# Autodesk Inventor assembly: ASY MSC 080 gills
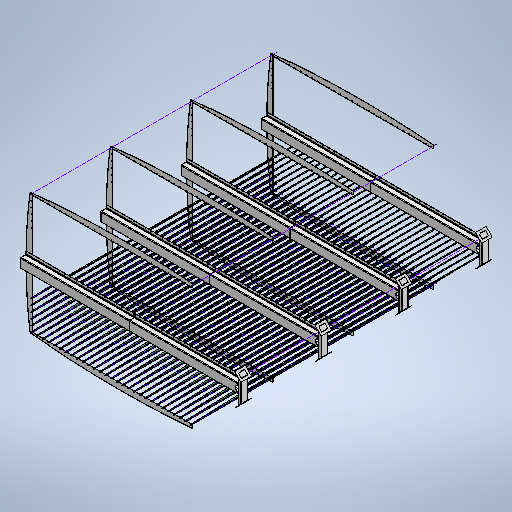
[picture p0: Inventor's stored thumbnail of the model, 512x512]
Saved by Autodesk Inventor 2025 (Build 290162010, 162A)
## iProperties
Created: 2024-08-31
Part Number: ASY MSC 080 gills
Document SubType Name: Assembly
Designer: pokla
Stock Number: ASY МОО 080 Жабры
Author: pokla
## Documents named in this file (20)
- C:\Users\admin\YandexDisk-badmisterfox\домашниий пк\Inventor\Manturovo\Manturovo_Se-clar\ASY MSC 080 gills.iam
- C:\Users\admin\YandexDisk-badmisterfox\домашниий пк\Inventor\Manturovo\Manturovo_Se-clar\MSC 802 sheet gills.ipt
- C:\Users\admin\YandexDisk-badmisterfox\домашниий пк\Inventor\Manturovo\Manturovo_Se-clar\MSC 081 pillar gills.ipt
- C:\Users\admin\YandexDisk-badmisterfox\домашниий пк\Inventor\Manturovo\Manturovo_Se-clar\MSC 804 sheet gills.ipt
- C:\Users\admin\YandexDisk-badmisterfox\домашниий пк\Inventor\Manturovo\Manturovo_Se-clar\MSC 803 sheet gills.ipt
- C:\Users\admin\YandexDisk-badmisterfox\домашниий пк\Inventor\Manturovo\Manturovo_Se-clar\MSC 806 sheet gills.ipt
- C:\Users\admin\YandexDisk-badmisterfox\домашниий пк\Inventor\Manturovo\Manturovo_Se-clar\MSC 805 sheet gills.ipt
- C:\Users\admin\YandexDisk-badmisterfox\домашниий пк\Inventor\Manturovo\Manturovo_Se-clar\MSC 808 sheet gills.ipt
- C:\Users\admin\YandexDisk-badmisterfox\домашниий пк\Inventor\Manturovo\Manturovo_Se-clar\MSC 807 sheet gills.ipt
- C:\Users\admin\YandexDisk-badmisterfox\домашниий пк\Inventor\Manturovo\Manturovo_Se-clar\MSC 810 sheet gills.ipt
- C:\Users\admin\YandexDisk-badmisterfox\домашниий пк\Inventor\Manturovo\Manturovo_Se-clar\MSC 809 sheet gills.ipt
- C:\Users\admin\YandexDisk-badmisterfox\домашниий пк\Inventor\Manturovo\Manturovo_Se-clar\MSC 812 sheet gills.ipt
- C:\Users\admin\YandexDisk-badmisterfox\домашниий пк\Inventor\Manturovo\Manturovo_Se-clar\MSC 811 sheet gills.ipt
- C:\Users\admin\YandexDisk-badmisterfox\домашниий пк\Inventor\Manturovo\Manturovo_Se-clar\MSC 084 wall support gills.ipt
- C:\Users\admin\YandexDisk-badmisterfox\домашниий пк\Inventor\Manturovo\Manturovo_Se-clar\MSC 085 bottom support gills.ipt
- C:\Users\admin\YandexDisk-badmisterfox\домашниий пк\Inventor\Manturovo\Manturovo_Se-clar\MSC 082 pillar gills.ipt
- C:\Users\admin\YandexDisk-badmisterfox\домашниий пк\Inventor\Manturovo\Manturovo_Se-clar\MSC 086 string for sheets gills.ipt
- C:\Users\admin\YandexDisk-badmisterfox\домашниий пк\Inventor\Manturovo\Manturovo_Se-clar\MSC 083 top support gills.ipt
- C:\Users\admin\YandexDisk-badmisterfox\домашниий пк\Inventor\Manturovo\Manturovo_Se-clar\MSC 087 bottom plate gills.ipt
- C:\Users\admin\YandexDisk-badmisterfox\домашниий пк\Inventor\Manturovo\Manturovo_Se-clar\MSC 801 sheet gills.ipt
## Components (175 placed, 19 different names)
1. MSC 804 sheet gills:1 — Rigid:39
2. MSC 803 sheet gills:1 — Angle:2, Tangent:8, Tangent:9, Flush:15, Flush:19, Rigid:39
3. MSC 806 sheet gills:1 — Rigid:36
4. MSC 805 sheet gills:1 — Rigid:36, Angle:3, Tangent:10, Tangent:11, Flush:15, Flush:16
5. MSC 808 sheet gills:1 — Rigid:37
6. MSC 807 sheet gills:1 — Rigid:37, Angle:4, Tangent:12, Tangent:13, Flush:16, Flush:17
7. MSC 810 sheet gills:1 — Rigid:38
8. MSC 809 sheet gills:1 — Rigid:38, Angle:5, Tangent:17, Tangent:18, Flush:17, Flush:18
9. MSC 812 sheet gills:1 — Rigid:32
10. MSC 811 sheet gills:1 — Rigid:32, Angle:6, Tangent:19, Tangent:20, Flush:18
11. MSC 084 wall support gills:1 — Rigid:12, Rigid:25, Rigid:30, Tangent:14, Tangent:15
12. MSC 084 wall support gills:2 — Rigid:25, Rigid:26, Mate:17
13. MSC 084 wall support gills:3 — Rigid:26, Rigid:27
14. MSC 084 wall support gills:4 — Rigid:27
15. MSC 086 string for sheets gills:2 — Rigid:15
16. MSC 086 string for sheets gills:57 — Rotational:2
17. MSC 085 bottom support gills:1 — Rigid:6, Rigid:7, Flush:12, Mate:12, Flush:14, Mate:15, Mate:16, Flush:9
18. MSC 081 pillar gills:1 — Flush:12, Mate:12, Flush:14, Rotational:1, Rotational:2, Tangent:16
19. MSC 082 pillar gills:1 — Rigid:28, Rigid:29
20. MSC 085 bottom support gills:2
21. MSC 081 pillar gills:2
22. MSC 082 pillar gills:2
23. MSC 085 bottom support gills:3
24. MSC 081 pillar gills:3
25. MSC 082 pillar gills:3
26. MSC 085 bottom support gills:4
27. MSC 081 pillar gills:4
28. MSC 082 pillar gills:4
29. MSC 801 sheet gills:1 — Mate:17, Rigid:33, Angle:2, Angle:3, Angle:4, Angle:5, Angle:6, Tangent:14, Tangent:15, Tangent:16, Flush:19
30. MSC 802 sheet gills:1 — Rigid:33
31. MSC 801 sheet gills:2
32. MSC 802 sheet gills:2
33. MSC 801 sheet gills:3
34. MSC 802 sheet gills:3
35. MSC 801 sheet gills:4
36. MSC 802 sheet gills:4
37. MSC 801 sheet gills:5
38. MSC 802 sheet gills:5
39. MSC 801 sheet gills:6
40. MSC 802 sheet gills:6
41. MSC 801 sheet gills:7
42. MSC 802 sheet gills:7
43. MSC 801 sheet gills:8
44. MSC 802 sheet gills:8
45. MSC 801 sheet gills:9
46. MSC 802 sheet gills:9
47. MSC 801 sheet gills:10
48. MSC 802 sheet gills:10
49. MSC 801 sheet gills:11
50. MSC 802 sheet gills:11
51. MSC 801 sheet gills:12
52. MSC 802 sheet gills:12
53. MSC 801 sheet gills:13
54. MSC 802 sheet gills:13
55. MSC 801 sheet gills:14
56. MSC 802 sheet gills:14
57. MSC 801 sheet gills:15
58. MSC 802 sheet gills:15
59. MSC 801 sheet gills:16
60. MSC 802 sheet gills:16
61. MSC 801 sheet gills:17
62. MSC 802 sheet gills:17
63. MSC 801 sheet gills:18
64. MSC 802 sheet gills:18
65. MSC 801 sheet gills:19
66. MSC 802 sheet gills:19
67. MSC 801 sheet gills:20
68. MSC 802 sheet gills:20
69. MSC 801 sheet gills:21
70. MSC 802 sheet gills:21
71. MSC 801 sheet gills:22
72. MSC 802 sheet gills:22
73. MSC 801 sheet gills:23
74. MSC 802 sheet gills:23
75. MSC 801 sheet gills:24
76. MSC 802 sheet gills:24
77. MSC 801 sheet gills:25
78. MSC 802 sheet gills:25
79. MSC 801 sheet gills:26
80. MSC 802 sheet gills:26
81. MSC 801 sheet gills:27
82. MSC 802 sheet gills:27
83. MSC 801 sheet gills:28
84. MSC 802 sheet gills:28
85. MSC 801 sheet gills:29
86. MSC 802 sheet gills:29
87. MSC 084 wall support gills:5 — Rigid:15, Rigid:31
88. MSC 083 top support gills:1 — Rigid:24, Rigid:29, Rigid:31
89. MSC 083 top support gills:2 — Rigid:28, Rigid:30, Tangent:8, Tangent:9, Tangent:10, Tangent:11, Tangent:12, Tangent:13, Tangent:17, Tangent:18, Tangent:19, Tangent:20, Rigid:40
90. MSC 087 bottom plate gills:1 — Rigid:6
91. MSC 087 bottom plate gills:2 — Rigid:7
92. MSC 084 wall support gills:6
93. MSC 083 top support gills:3
94. MSC 083 top support gills:4
95. MSC 087 bottom plate gills:3
96. MSC 087 bottom plate gills:4
97. MSC 084 wall support gills:7
98. MSC 083 top support gills:5
99. MSC 083 top support gills:6
100. MSC 087 bottom plate gills:5
101. MSC 087 bottom plate gills:6
102. MSC 084 wall support gills:8
103. MSC 083 top support gills:7
104. MSC 083 top support gills:8
105. MSC 087 bottom plate gills:7
106. MSC 087 bottom plate gills:8
107. MSC 086 string for sheets gills:1 — Rigid:12
108. MSC 086 string for sheets gills:3
109. MSC 086 string for sheets gills:5
110. MSC 086 string for sheets gills:7
111. MSC 086 string for sheets gills:9
112. MSC 086 string for sheets gills:11
113. MSC 086 string for sheets gills:13
114. MSC 086 string for sheets gills:15
115. MSC 086 string for sheets gills:17
116. MSC 086 string for sheets gills:19
117. MSC 086 string for sheets gills:21
118. MSC 086 string for sheets gills:23
119. MSC 086 string for sheets gills:25
120. MSC 086 string for sheets gills:27
121. MSC 086 string for sheets gills:29
122. MSC 086 string for sheets gills:31
123. MSC 086 string for sheets gills:33
124. MSC 086 string for sheets gills:35
125. MSC 086 string for sheets gills:37
126. MSC 086 string for sheets gills:39
127. MSC 086 string for sheets gills:41
128. MSC 086 string for sheets gills:43
129. MSC 086 string for sheets gills:45
130. MSC 086 string for sheets gills:47
131. MSC 086 string for sheets gills:49
132. MSC 086 string for sheets gills:51
133. MSC 086 string for sheets gills:53
134. MSC 086 string for sheets gills:55
135. MSC 086 string for sheets gills:58 — Rotational:1
136. MSC 086 string for sheets gills:60
137. MSC 086 string for sheets gills:62
138. MSC 086 string for sheets gills:64
139. MSC 086 string for sheets gills:66
140. MSC 086 string for sheets gills:68
141. MSC 086 string for sheets gills:70
142. MSC 086 string for sheets gills:72
143. MSC 086 string for sheets gills:74
144. MSC 086 string for sheets gills:76
145. MSC 086 string for sheets gills:78
146. MSC 086 string for sheets gills:80
147. MSC 086 string for sheets gills:82
148. MSC 086 string for sheets gills:84
149. MSC 086 string for sheets gills:86
150. MSC 086 string for sheets gills:88
151. MSC 086 string for sheets gills:90
152. MSC 086 string for sheets gills:92
153. MSC 086 string for sheets gills:94
154. MSC 086 string for sheets gills:96
155. MSC 086 string for sheets gills:98
156. MSC 086 string for sheets gills:100
157. MSC 086 string for sheets gills:102
158. MSC 086 string for sheets gills:104
159. MSC 086 string for sheets gills:106
160. MSC 086 string for sheets gills:108
161. MSC 086 string for sheets gills:110
162. MSC 086 string for sheets gills:112
163. MSC 086 string for sheets gills:114
164. MSC 086 string for sheets gills:116
165. MSC 086 string for sheets gills:118
166. MSC 086 string for sheets gills:120
167. MSC 086 string for sheets gills:122
168. MSC 086 string for sheets gills:124
169. MSC 086 string for sheets gills:125 — Rigid:40
170. MSC 086 string for sheets gills:126
171. MSC 086 string for sheets gills:127
172. MSC 086 string for sheets gills:128
173. MSC 086 string for sheets gills:129
174. MSC 086 string for sheets gills:130
175. MSC 086 string for sheets gills:131 — Rigid:24
## Component patterns: (4 elements, first: MSC 085 bottom support gills:1 + MSC 081 pillar gills:1 + MSC 082 pillar gills:1), (29 elements, first: MSC 801 sheet gills:1 + MSC 802 sheet gills:1), (4 elements, first: MSC 084 wall support gills:5 + MSC 083 top support gills:1 + MSC 083 top support gills:2 + MSC 087 bottom plate gills:1 + MSC 087 bottom plate gills:2), (28 elements, first: MSC 086 string for sheets gills:1), (34 elements, first: MSC 086 string for sheets gills:58), (6 elements, first: MSC 086 string for sheets gills:125), (1 elements, first: MSC 086 string for sheets gills:131)
## Relationships (52: WeldJoint 20, Tangent 13, Flush 8, Angle 5, Mate 4, RevoluteJoint 2)
- [WeldJoint]: MSC 081 pillar gills:1 ↔ MSC 082 pillar gills:1
- Rigid:6 [WeldJoint]: MSC 085 bottom support gills:1 ↔ MSC 087 bottom plate gills:1
- Rigid:7 [WeldJoint]: MSC 085 bottom support gills:1 ↔ MSC 087 bottom plate gills:2
- Flush:12: MSC 085 bottom support gills:1 ↔ MSC 081 pillar gills:1
- Mate:12: MSC 085 bottom support gills:1 ↔ MSC 081 pillar gills:1
- Flush:14 (5 mm): MSC 085 bottom support gills:1 ↔ MSC 081 pillar gills:1
- Rigid:12 [WeldJoint] (-5 mm): MSC 084 wall support gills:1 ↔ MSC 086 string for sheets gills:1
- Rigid:15 [WeldJoint] (-5 mm): MSC 086 string for sheets gills:2 ↔ MSC 084 wall support gills:5
- Mate:15: MSC 085 bottom support gills:1
- Mate:16: MSC 085 bottom support gills:1
- Flush:9: MSC 085 bottom support gills:1
- Rigid:24 [WeldJoint] (-5 mm): MSC 083 top support gills:1 ↔ MSC 086 string for sheets gills:131
- Rigid:25 [WeldJoint] (985 mm): MSC 084 wall support gills:1 ↔ MSC 084 wall support gills:2
- Rigid:26 [WeldJoint] (985 mm): MSC 084 wall support gills:2 ↔ MSC 084 wall support gills:3
- Rigid:27 [WeldJoint] (985 mm): MSC 084 wall support gills:3 ↔ MSC 084 wall support gills:4
- Mate:17: MSC 084 wall support gills:2 ↔ MSC 801 sheet gills:1
- Rigid:28 [WeldJoint]: MSC 082 pillar gills:1 ↔ MSC 083 top support gills:2
- Rigid:29 [WeldJoint]: MSC 082 pillar gills:1 ↔ MSC 083 top support gills:1
- Rigid:30 [WeldJoint]: MSC 084 wall support gills:1 ↔ MSC 083 top support gills:2
- Rigid:31 [WeldJoint]: MSC 084 wall support gills:5 ↔ MSC 083 top support gills:1
- Rotational:1 [RevoluteJoint] (5 mm): MSC 081 pillar gills:1 ↔ MSC 086 string for sheets gills:58
- Rotational:2 [RevoluteJoint] (-5 mm): MSC 086 string for sheets gills:57 ↔ MSC 081 pillar gills:1
- Rigid:32 [WeldJoint] (-10 mm): MSC 812 sheet gills:1 ↔ MSC 811 sheet gills:1
- Rigid:33 [WeldJoint] (-10 mm): MSC 801 sheet gills:1 ↔ MSC 802 sheet gills:1
- Rigid:36 [WeldJoint] (-10 mm): MSC 806 sheet gills:1 ↔ MSC 805 sheet gills:1
- Rigid:37 [WeldJoint] (-10 mm): MSC 808 sheet gills:1 ↔ MSC 807 sheet gills:1
- Rigid:38 [WeldJoint] (-10 mm): MSC 810 sheet gills:1 ↔ MSC 809 sheet gills:1
- Angle:2 (0 deg): MSC 803 sheet gills:1 ↔ MSC 801 sheet gills:1
- Angle:3 (0 deg): MSC 805 sheet gills:1 ↔ MSC 801 sheet gills:1
- Angle:4 (0 deg): MSC 807 sheet gills:1 ↔ MSC 801 sheet gills:1
- Angle:5 (0 deg): MSC 809 sheet gills:1 ↔ MSC 801 sheet gills:1
- Angle:6 (0 deg): MSC 811 sheet gills:1 ↔ MSC 801 sheet gills:1
- Tangent:8: MSC 803 sheet gills:1 ↔ MSC 083 top support gills:2
- Tangent:9: MSC 803 sheet gills:1 ↔ MSC 083 top support gills:2
- Tangent:10: MSC 805 sheet gills:1 ↔ MSC 083 top support gills:2
- Tangent:11: MSC 805 sheet gills:1 ↔ MSC 083 top support gills:2
- Tangent:12: MSC 807 sheet gills:1 ↔ MSC 083 top support gills:2
- Tangent:13: MSC 807 sheet gills:1 ↔ MSC 083 top support gills:2
- Tangent:14: MSC 084 wall support gills:1 ↔ MSC 801 sheet gills:1
- Tangent:15: MSC 084 wall support gills:1 ↔ MSC 801 sheet gills:1
- Tangent:16: MSC 081 pillar gills:1 ↔ MSC 801 sheet gills:1
- Tangent:17: MSC 809 sheet gills:1 ↔ MSC 083 top support gills:2
- Tangent:18: MSC 809 sheet gills:1 ↔ MSC 083 top support gills:2
- Tangent:19: MSC 811 sheet gills:1 ↔ MSC 083 top support gills:2
- Tangent:20: MSC 811 sheet gills:1 ↔ MSC 083 top support gills:2
- Flush:15: MSC 803 sheet gills:1 ↔ MSC 805 sheet gills:1
- Flush:16: MSC 805 sheet gills:1 ↔ MSC 807 sheet gills:1
- Flush:17: MSC 807 sheet gills:1 ↔ MSC 809 sheet gills:1
- Flush:18: MSC 809 sheet gills:1 ↔ MSC 811 sheet gills:1
- Flush:19: MSC 803 sheet gills:1 ↔ MSC 801 sheet gills:1
- Rigid:39 [WeldJoint] (-10 mm): MSC 804 sheet gills:1 ↔ MSC 803 sheet gills:1
- Rigid:40 [WeldJoint] (5 mm): MSC 083 top support gills:2 ↔ MSC 086 string for sheets gills:125
